# Autodesk Inventor assembly: leg_2
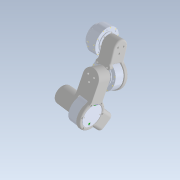
[picture p0: Inventor's stored thumbnail of the model, 180x180]
Saved by Autodesk Inventor 2020 (Build 240168000, 168)
## iProperties
Created: 2021-01-03
Part Number: leg_2
Document SubType Name: Assembly
Designer: DELL
Author: DELL
## Documents named in this file (6)
- F:\SoftRobot2.0\Flexipod2.0\robot_2021_1_3\leg_2.iam
- F:\SoftRobot2.0\Flexipod2.0\RMD_X6_stator.ipt
- F:\SoftRobot2.0\Flexipod2.0\RMD_X6_rotor.ipt
- F:\SoftRobot2.0\Flexipod2.0\robot_2021_1_3\hip_link_2.ipt
- F:\SoftRobot2.0\Flexipod2.0\robot_2021_1_3\thigh_link_2.ipt
- F:\SoftRobot2.0\Flexipod2.0\robot_2021_1_3\shank_link.ipt
## Components (9 placed, 5 different names)
1. RMD_X6_stator:1 — Mate:1, Flush:1
2. RMD_X6_rotor:1 — Mate:1, Flush:1, Mate:2, Mate:3, Mate:4
3. hip_link_2:1 — Mate:2, Mate:3, Mate:4, Mate:6, Mate:7, Mate:8
4. RMD_X6_stator:2 — Mate:6, Mate:7, Mate:8, Mate:10
5. RMD_X6_rotor:2 — Mate:11, Mate:12
6. RMD_X6_stator:3 — Mate:13, Mate:14, Mate:15, Mate:16
7. RMD_X6_rotor:3 — Mate:17, Mate:18
8. thigh_link_2:1 — Mate:10, Mate:11, Mate:12, Mate:13, Mate:14, Mate:15
9. shank_link:1 — Mate:16, Mate:17, Mate:18
## Relationships (21: Mate 18, Flush 3)
- Mate:1: RMD_X6_stator:1 ↔ RMD_X6_rotor:1
- Flush:1 (-3 mm): RMD_X6_stator:1 ↔ RMD_X6_rotor:1
- Mate:2: RMD_X6_rotor:1 ↔ hip_link_2:1
- Mate:3: RMD_X6_rotor:1 ↔ hip_link_2:1
- Mate:4: RMD_X6_rotor:1 ↔ hip_link_2:1
- [Mate]: RMD_X6_stator:2 ↔ RMD_X6_rotor:2
- [Flush] (-3 mm): RMD_X6_stator:2 ↔ RMD_X6_rotor:2
- Mate:6: hip_link_2:1 ↔ RMD_X6_stator:2
- Mate:7: hip_link_2:1 ↔ RMD_X6_stator:2
- Mate:8: hip_link_2:1 ↔ RMD_X6_stator:2
- [Mate]: RMD_X6_stator:3 ↔ RMD_X6_rotor:3
- [Flush] (-3 mm): RMD_X6_stator:3 ↔ RMD_X6_rotor:3
- Mate:10: RMD_X6_stator:2 ↔ thigh_link_2:1
- Mate:11: RMD_X6_rotor:2 ↔ thigh_link_2:1
- Mate:12: RMD_X6_rotor:2 ↔ thigh_link_2:1
- Mate:13: RMD_X6_stator:3 ↔ thigh_link_2:1
- Mate:14: RMD_X6_stator:3 ↔ thigh_link_2:1
- Mate:15: RMD_X6_stator:3 ↔ thigh_link_2:1
- Mate:16: RMD_X6_stator:3 ↔ shank_link:1
- Mate:17: RMD_X6_rotor:3 ↔ shank_link:1
- Mate:18: RMD_X6_rotor:3 ↔ shank_link:1
## Named parameters: d5_d0 = 0 mm, d6_d1 = -3 mm, d10_d5_d0 = 0 mm, d11_d6_d1 = -3 mm
